# Autodesk Inventor assembly: midi_splitter
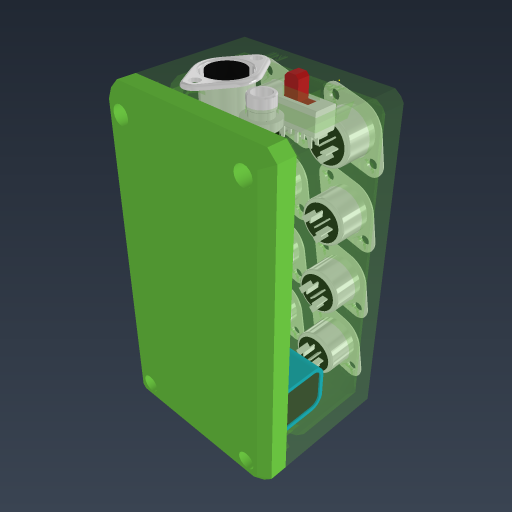
[picture p0: Inventor's stored thumbnail of the model, 512x512]
Saved by Autodesk Inventor 2024 (Build 280153000, 153)
## iProperties
Created: 2020-11-28
Part Number: midi_splitter
Document SubType Name: Assembly
Designer: Milosz
Author: Milosz
## Documents named in this file (8)
- E:\Projekty\Glowne\MidiSplitter\mechanics\midi_splitter.iam
- E:\Projekty\Glowne\MidiSplitter\mechanics\Case1.ipt
- E:\Projekty\Glowne\MidiSplitter\mechanics\gniazdo_zasilania.ipt
- E:\Projekty\Glowne\MidiSplitter\mechanics\midi_gniazdo.ipt
- E:\Projekty\Glowne\MidiSplitter\mechanics\Case2.ipt
- E:\Projekty\Glowne\MidiSplitter\mechanics\PCB\MIDI Splitter.iam
- E:\Projekty\Glowne\MidiSplitter\mechanics\battery_holder\9-volt-battery-2.snapshot.6\Battery\Battery_updated.ipt
- E:\Projekty\Glowne\MidiSplitter\mechanics\switch.ipt
## Components (15 placed, 7 different names)
1. Case1:1 — Mate:1, Mate:2, Mate:3, Mate:4, Mate:5, Mate:6, Mate:7, Mate:8, Mate:9, Mate:10, Mate:11, Mate:12, Mate:13, Mate:14, Mate:15, Mate:16, Mate:17, Mate:18, Mate:20, Mate:21, Mate:23, Mate:25, Mate:26, Mate:27, Mate:28, Mate:29, Mate:30, Mate:31, Mate:39, Mate:40, Mate:41, Mate:42
2. gniazdo_zasilania:1 — Mate:30, Mate:31
3. midi_gniazdo:1 — Mate:23, Mate:25, Mate:26
4. midi_gniazdo:2 — Flush:2, Mate:9, Mate:10
5. midi_gniazdo:3 — Flush:2, Flush:3, Mate:7, Mate:8
6. midi_gniazdo:4 — Flush:3, Flush:4, Mate:1, Mate:2, Mate:3, Mate:4
7. midi_gniazdo:5 — Flush:4, Flush:5, Flush:6, Mate:11, Mate:12
8. midi_gniazdo:6 — Flush:7, Mate:15, Mate:16
9. midi_gniazdo:7 — Flush:8, Mate:17, Mate:18
10. midi_gniazdo:8 — Flush:6, Flush:7, Flush:8, Mate:13, Mate:14
11. midi_gniazdo:9 — Flush:5, Mate:5, Mate:6
12. Case2:1 — Mate:20, Mate:21, Mate:27, Mate:28, Mate:29, Mate:32, Mate:33, Mate:34, Mate:38, Mate:39
13. MIDI Splitter:1 [sub-assembly] — Mate:32, Mate:33, Mate:34
14. Battery_updated:1 — Mate:38
15. switch:1 — Mate:40, Mate:41, Mate:42
## Relationships (43: Mate 36, Flush 7)
- Flush:2: midi_gniazdo:2 ↔ midi_gniazdo:3
- Flush:3: midi_gniazdo:3 ↔ midi_gniazdo:4
- Flush:4: midi_gniazdo:4 ↔ midi_gniazdo:5
- Flush:5: midi_gniazdo:5 ↔ midi_gniazdo:9
- Flush:6: midi_gniazdo:5 ↔ midi_gniazdo:8
- Flush:7: midi_gniazdo:6 ↔ midi_gniazdo:8
- Flush:8: midi_gniazdo:7 ↔ midi_gniazdo:8
- Mate:1: Case1:1 ↔ midi_gniazdo:4
- Mate:2: Case1:1 ↔ midi_gniazdo:4
- Mate:3: Case1:1 ↔ midi_gniazdo:4
- Mate:4: Case1:1 ↔ midi_gniazdo:4
- Mate:5: Case1:1 ↔ midi_gniazdo:9
- Mate:6: Case1:1 ↔ midi_gniazdo:9
- Mate:7: Case1:1 ↔ midi_gniazdo:3
- Mate:8: Case1:1 ↔ midi_gniazdo:3
- Mate:9: Case1:1 ↔ midi_gniazdo:2
- Mate:10: Case1:1 ↔ midi_gniazdo:2
- Mate:11: Case1:1 ↔ midi_gniazdo:5
- Mate:12: Case1:1 ↔ midi_gniazdo:5
- Mate:13: Case1:1 ↔ midi_gniazdo:8
- Mate:14: Case1:1 ↔ midi_gniazdo:8
- Mate:15: Case1:1 ↔ midi_gniazdo:6
- Mate:16: Case1:1 ↔ midi_gniazdo:6
- Mate:17: Case1:1 ↔ midi_gniazdo:7
- Mate:18: Case1:1 ↔ midi_gniazdo:7
- Mate:20: Case1:1 ↔ Case2:1
- Mate:21: Case1:1 ↔ Case2:1
- Mate:23: Case1:1 ↔ midi_gniazdo:1
- Mate:25: Case1:1 ↔ midi_gniazdo:1
- Mate:26: Case1:1 ↔ midi_gniazdo:1
- Mate:27: Case1:1 ↔ Case2:1
- Mate:28: Case1:1 ↔ Case2:1
- Mate:29: Case1:1 ↔ Case2:1
- Mate:30: Case1:1 ↔ gniazdo_zasilania:1
- Mate:31: Case1:1 ↔ gniazdo_zasilania:1
- Mate:32: Case2:1 ↔ MIDI Splitter:1
- Mate:33: Case2:1 ↔ MIDI Splitter:1
- Mate:34: Case2:1 ↔ MIDI Splitter:1
- Mate:38: Case2:1 ↔ Battery_updated:1
- Mate:39: Case1:1 ↔ Case2:1
- Mate:40: Case1:1 ↔ switch:1
- Mate:41: Case1:1 ↔ switch:1
- Mate:42: Case1:1 ↔ switch:1
